# Autodesk Inventor assembly: structure
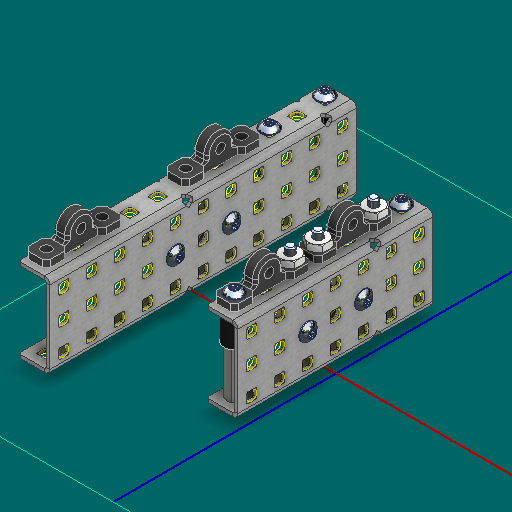
[picture p0: Inventor's stored thumbnail of the model, 512x512]
Saved by Autodesk Inventor 2025 (Build 290162000, 162)
## iProperties
Created: 2024-08-16
Part Number: structure
Document SubType Name: Assembly
Designer: averey
Author: averey
## Documents named in this file (22)
- C:\Users\avere\vex_robotics_high_stakes\hardware\cad\ATLAS\chassis\drive_pod\back_left\structure.iam
- C:\Users\avere\vex_robotics_high_stakes\hardware\cad\VEX-CAD-Inventor\Structure\C Channel\Aluminum 1x3x1\Alu C 1x3x1x7.ipt
- C:\Users\avere\vex_robotics_high_stakes\hardware\cad\_quick_assemblies\bearing_flat_w_hardware.iam
- C:\Users\avere\vex_robotics_high_stakes\hardware\cad\VEX-CAD-Inventor\Structure\C Channel\Aluminum 1x3x1\Alu C 1x3x1x11.ipt
- C:\Users\avere\vex_robotics_high_stakes\hardware\cad\VEX-CAD-Inventor\Motion\Shaft LS\LS Pillow Bearing Block.ipt
- C:\Users\avere\vex_robotics_high_stakes\hardware\cad\VEX-CAD-Inventor\Motion\Spacers\Spacer Nylon .375 OD.ipt
- C:\Users\avere\vex_robotics_high_stakes\hardware\cad\VEX-CAD-Inventor\Motion\Spacers\Spacer Nylon .375 OD\NSpacer .375 OD x .500.ipt
- C:\Users\avere\vex_robotics_high_stakes\hardware\cad\VEX-CAD-Inventor\Structure\Standoff\Standoff .875.ipt
- C:\Users\avere\vex_robotics_high_stakes\hardware\cad\VEX-CAD-Inventor\Structure\Standoff.ipt
- C:\Users\avere\vex_robotics_high_stakes\hardware\cad\VEX-CAD-Inventor\Structure\Hardware\Screw Shoulder Robosource\SScrew Shoulder Smooth .375 x .12.ipt
- C:\Users\avere\vex_robotics_high_stakes\hardware\cad\VEX-CAD-Inventor\Structure\Hardware\Screw Shoulder Robosource.ipt
- C:\Users\avere\vex_robotics_high_stakes\hardware\cad\VEX-CAD-Inventor\Structure\Hardware\Screw Steel - Star\SScrew Star Smooth .875.ipt
- C:\Users\avere\vex_robotics_high_stakes\hardware\cad\VEX-CAD-Inventor\Structure\Hardware\Screw Steel - Star.ipt
- C:\Users\avere\vex_robotics_high_stakes\hardware\cad\VEX-CAD-Inventor\Structure\Hardware\Screw Shoulder Robosource\SScrew Shoulder Smooth .500 x .18.ipt
- C:\Users\avere\vex_robotics_high_stakes\hardware\cad\VEX-CAD-Inventor\Structure\Hardware\Nut Nylon\Nut Nylon - White.ipt
- C:\Users\avere\vex_robotics_high_stakes\hardware\cad\VEX-CAD-Inventor\Structure\Hardware\Nut Nylon.ipt
- C:\Users\avere\vex_robotics_high_stakes\hardware\cad\VEX-CAD-Inventor\Structure\Standoff\Standoff 1.25.ipt
- C:\Users\avere\vex_robotics_high_stakes\hardware\cad\VEX-CAD-Inventor\Motion\Spacers\Washer Steel\SWasher .375 OD x .062500.ipt
- C:\Users\avere\vex_robotics_high_stakes\hardware\cad\VEX-CAD-Inventor\Motion\Spacers\Washer Steel.ipt
- C:\Users\avere\vex_robotics_high_stakes\hardware\cad\VEX-CAD-Inventor\Structure\Standoff\Standoff 1.00.ipt
- C:\Users\avere\vex_robotics_high_stakes\hardware\cad\VEX-CAD-Inventor\Motion\Spacers\Spacer Nylon .375 OD\NSpacer .375 OD x .125.ipt
- C:\Users\avere\vex_robotics_high_stakes\hardware\cad\VEX-CAD-Inventor\Structure\Hardware\Screw Shoulder Robosource\SScrew Shoulder Smooth .500 x .04.ipt
## Components (32 placed, 15 different names)
1. Alu C 1x3x1x7:1 — Mate:1, Insert:1, Mate:2, Insert:2, Mate:3, Insert:4, Mate:5, Insert:5, Mate:6, Insert:15, Insert:16, Insert:18, Insert:21, Insert:24, Insert:25, Insert:26, Insert:27
2. bearing_flat_w_hardware:1 [sub-assembly] — Insert:1, Mate:2
3. Alu C 1x3x1x11:1 — Insert:2, Mate:3, Insert:3, Mate:4, Insert:6, Mate:7, Insert:7, Mate:8, Insert:31, Insert:35, Insert:37, Insert:38, Insert:40, Insert:41
4. bearing_flat_w_hardware:2 [sub-assembly] — Insert:3, Mate:4
5. LS Pillow Bearing Block:1 — Insert:4, Mate:5, Insert:17, Insert:19
6. LS Pillow Bearing Block:2 — Insert:5, Mate:6, Insert:20, Insert:28
7. LS Pillow Bearing Block:3 — Insert:6, Mate:7
8. LS Pillow Bearing Block:4 — Insert:7, Mate:8
9. NSpacer .375 OD x .500:7 — Insert:14
10. Standoff .875:1 — Insert:14, Insert:15
11. SScrew Shoulder Smooth .375 x .12:1 — Insert:16
12. SScrew Star Smooth .875:1 — Insert:17
13. SScrew Shoulder Smooth .500 x .18:2 — Insert:18
14. Nut Nylon - White:1 — Insert:19
15. SScrew Shoulder Smooth .500 x .18:3 — Insert:21
16. Nut Nylon - White:2 — Insert:20
17. Standoff 1.25:1 — Insert:22, Insert:23
18. SWasher .375 OD x .062500:1 — Insert:22, Insert:24
19. SWasher .375 OD x .062500:2 — Insert:23
20. SScrew Shoulder Smooth .500 x .18:4 — Insert:26
21. SScrew Shoulder Smooth .500 x .18:5 — Insert:25
22. SScrew Shoulder Smooth .500 x .18:6 — Insert:27
23. Nut Nylon - White:3 — Insert:28
24. Standoff 1.25:2
25. SWasher .375 OD x .062500:3
26. SWasher .375 OD x .062500:4 — Insert:31
27. SScrew Shoulder Smooth .500 x .18:7 — Insert:38
28. SScrew Shoulder Smooth .500 x .18:9 — Insert:37
29. SScrew Shoulder Smooth .500 x .18:10 — Insert:35
30. Standoff 1.00:2 — Insert:39
31. NSpacer .375 OD x .125:8 — Insert:39, Insert:40
32. SScrew Shoulder Smooth .500 x .04:11 — Insert:41
## Relationships (39: Insert 31, Mate 8)
- Mate:1: Alu C 1x3x1x7:1
- Insert:1: Alu C 1x3x1x7:1 ↔ bearing_flat_w_hardware:1
- Mate:2: Alu C 1x3x1x7:1 ↔ bearing_flat_w_hardware:1
- Insert:2 (58.7375 mm): Alu C 1x3x1x7:1 ↔ Alu C 1x3x1x11:1
- Mate:3: Alu C 1x3x1x7:1 ↔ Alu C 1x3x1x11:1
- Insert:3: Alu C 1x3x1x11:1 ↔ bearing_flat_w_hardware:2
- Mate:4: Alu C 1x3x1x11:1 ↔ bearing_flat_w_hardware:2
- Insert:4 (1.5875 mm): Alu C 1x3x1x7:1 ↔ LS Pillow Bearing Block:1
- Mate:5: Alu C 1x3x1x7:1 ↔ LS Pillow Bearing Block:1
- Insert:5 (1.5875 mm): Alu C 1x3x1x7:1 ↔ LS Pillow Bearing Block:2
- Mate:6: Alu C 1x3x1x7:1 ↔ LS Pillow Bearing Block:2
- Insert:6 (1.5875 mm): Alu C 1x3x1x11:1 ↔ LS Pillow Bearing Block:3
- Mate:7: Alu C 1x3x1x11:1 ↔ LS Pillow Bearing Block:3
- Insert:7 (1.5875 mm): Alu C 1x3x1x11:1 ↔ LS Pillow Bearing Block:4
- Mate:8: Alu C 1x3x1x11:1 ↔ LS Pillow Bearing Block:4
- Insert:14: NSpacer .375 OD x .500:7 ↔ Standoff .875:1
- Insert:15: Alu C 1x3x1x7:1 ↔ Standoff .875:1
- Insert:16 (1.5875 mm): Alu C 1x3x1x7:1 ↔ SScrew Shoulder Smooth .375 x .12:1
- Insert:17: LS Pillow Bearing Block:1 ↔ SScrew Star Smooth .875:1
- Insert:18: Alu C 1x3x1x7:1 ↔ SScrew Shoulder Smooth .500 x .18:2
- Insert:19: LS Pillow Bearing Block:1 ↔ Nut Nylon - White:1
- Insert:20: LS Pillow Bearing Block:2 ↔ Nut Nylon - White:2
- Insert:21: Alu C 1x3x1x7:1 ↔ SScrew Shoulder Smooth .500 x .18:3
- Insert:22: Standoff 1.25:1 ↔ SWasher .375 OD x .062500:1
- Insert:23: Standoff 1.25:1 ↔ SWasher .375 OD x .062500:2
- Insert:24: Alu C 1x3x1x7:1 ↔ SWasher .375 OD x .062500:1
- Insert:25 (1.5875 mm): Alu C 1x3x1x7:1 ↔ SScrew Shoulder Smooth .500 x .18:5
- Insert:26 (1.5875 mm): Alu C 1x3x1x7:1 ↔ SScrew Shoulder Smooth .500 x .18:4
- Insert:27: Alu C 1x3x1x7:1 ↔ SScrew Shoulder Smooth .500 x .18:6
- Insert:28: LS Pillow Bearing Block:2 ↔ Nut Nylon - White:3
- [Insert]: Standoff 1.25:2 ↔ SWasher .375 OD x .062500:3
- [Insert]: Standoff 1.25:2 ↔ SWasher .375 OD x .062500:4
- Insert:31: Alu C 1x3x1x11:1 ↔ SWasher .375 OD x .062500:4
- Insert:35 (1.5875 mm): Alu C 1x3x1x11:1 ↔ SScrew Shoulder Smooth .500 x .18:10
- Insert:37 (1.5875 mm): Alu C 1x3x1x11:1 ↔ SScrew Shoulder Smooth .500 x .18:9
- Insert:38 (1.5875 mm): Alu C 1x3x1x11:1 ↔ SScrew Shoulder Smooth .500 x .18:7
- Insert:39: Standoff 1.00:2 ↔ NSpacer .375 OD x .125:8
- Insert:40: Alu C 1x3x1x11:1 ↔ NSpacer .375 OD x .125:8
- Insert:41 (1.5875 mm): Alu C 1x3x1x11:1 ↔ SScrew Shoulder Smooth .500 x .04:11
## Named parameters: d40_d33 = 0 mm, d41_d34 = 0 mm
